# Autodesk Inventor assembly: x_motor
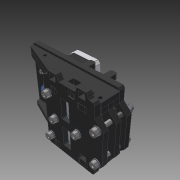
[picture p0: Inventor's stored thumbnail of the model, 180x180]
Saved by Autodesk Inventor 2014 (Build 180170000, 170)
## iProperties
Created: 2014-03-19
Part Number: x_motor
Document SubType Name: Assembly
Designer: buben
Author: buben
## Documents named in this file (18)
- C:\Users\buben\Documents\GitHub\bacon\inventor files\printer parts\6.5 mm\x_motor.iam
- C:\Users\buben\Documents\GitHub\bacon\inventor files\printer parts\6.5 mm\x_motor_back.ipt
- C:\Users\buben\Documents\GitHub\bacon\inventor files\printer parts\6.5 mm\motor_spacer.ipt
- C:\Users\buben\Documents\GitHub\bacon\inventor files\3rd party components\nema_17_stepper\Imported Components\NEMA 17 with T5 Pulley\NEMA 17 with T5 Pulley.iam
- C:\Users\buben\Documents\Inventor\Content Center Files\R2014\en-US\ISO 4762(2)\ISO 4762 - M3 x 16ISO.ipt
- C:\Users\buben\Documents\GitHub\bacon\inventor files\utils\washer_m3.ipt
- C:\Users\buben\Documents\GitHub\bacon\inventor files\printer parts\6.5 mm\x_motor_cable_mount.ipt
- C:\Users\buben\Documents\GitHub\bacon\inventor files\printer parts\6.5 mm\x_motor_cable_mount_brace.ipt
- C:\Users\buben\Documents\GitHub\bacon\inventor files\printer parts\6.5 mm\x_motor_smooth_rod_spacer.ipt
- C:\Users\buben\Documents\GitHub\bacon\inventor files\printer parts\6.5 mm\x_motor_wall_lower.ipt
- C:\Users\buben\Documents\GitHub\bacon\inventor files\printer parts\6.5 mm\x_motor_wall_upper.ipt
- C:\Users\buben\Documents\GitHub\bacon\inventor files\printer parts\6.5 mm\x_motor_middle.ipt
- C:\Users\buben\Documents\GitHub\bacon\inventor files\printer parts\6.5 mm\x_motor_upper_nut_stop.ipt
- C:\Users\buben\Documents\GitHub\bacon\inventor files\3rd party components\linear_bearing_8\Imported Components\LU8MM\LU8MM.iam
- C:\Users\buben\Documents\GitHub\bacon\inventor files\printer parts\6.5 mm\x_motor_top.ipt
- C:\Users\buben\Documents\GitHub\bacon\inventor files\utils\washer_m5.ipt
- C:\Users\buben\Documents\Inventor\Content Center Files\R2014\en-US\ISO 4762(2)\ISO 4762 - M5 x 45ISO.ipt
- C:\Users\buben\Documents\Inventor\Content Center Files\R2014\en-US\ISO 7040\ISO 7040 - M5.ipt
## Components (46 placed, 17 different names)
1. x_motor_back:1 — Mate:4, Tangent:1, Mate:5, Mate:6, Mate:7, Tangent:2, Mate:8, Mate:9, Mate:10, Mate:11, Mate:16, Mate:17, Mate:18, Mate:20, Mate:22, Mate:23, Mate:24, Mate:25, Mate:26, Mate:27, Mate:28, Mate:29, Mate:30, Mate:31, Mate:32, Mate:33, Mate:37, Mate:39, Mate:61, Mate:62, Mate:63, Mate:64, Mate:65, Mate:66
2. motor_spacer:1 — Mate:1, Mate:2, Mate:3, Mate:4, Tangent:1, Tangent:2, Mate:12, Mate:13, Mate:14, Mate:15
3. NEMA 17 with T5 Pulley:1 [sub-assembly] — Mate:1, Mate:2, Mate:3
4. ISO 4762 M3 x 16:1 — Insert:1, Mate:13
5. ISO 4762 M3 x 16:2 — Insert:2, Mate:12
6. ISO 4762 M3 x 16:3 — Insert:3, Mate:15
7. ISO 4762 M3 x 16:4 — Insert:4, Mate:14
8. CSN 02 1702 B B 3,2:1 — Mate:11, Insert:4
9. CSN 02 1702 B B 3,2:2 — Mate:10, Insert:3
10. CSN 02 1702 B B 3,2:3 — Mate:9, Insert:1
11. CSN 02 1702 B B 3,2:4 — Mate:8, Insert:2
12. x_motor_cable_mount:1 — Mate:16, Mate:17, Mate:18, Mate:19, Mate:21
13. x_motor_cable_mount_brace:1 — Mate:19, Mate:20, Mate:21
14. x_motor_smooth_rod_spacer:1 — Mate:23, Mate:24, Mate:27
15. x_motor_smooth_rod_spacer:2 — Mate:22, Mate:25, Mate:26
16. x_motor_wall_lower:1 — Mate:28, Mate:29, Mate:30, Mate:34, Mate:35, Mate:36, Mate:46, Mate:47
17. x_motor_wall_upper:1 — Mate:31, Mate:32, Mate:33, Mate:38
18. x_motor_middle:1 — Mate:34, Mate:35, Mate:36, Mate:40, Mate:41, Mate:42, Mate:43, Mate:44, Mate:45
19. x_motor_upper_nut_stop:1 — Mate:37, Mate:38, Mate:39
20. LU8MM:1 [sub-assembly] — Mate:40, Mate:41, Mate:45, Mate:48
21. LU8MM:2 [sub-assembly] — Mate:42, Mate:43, Mate:44
22. x_motor_top:1 — Mate:46, Mate:47, Mate:48, Mate:49, Mate:50, Mate:51, Mate:52, Mate:53, Mate:54, Mate:55, Mate:56, Mate:57, Mate:58, Mate:59, Mate:60
23. CSN 02 1702 B B 5,3:1 — Mate:53, Mate:56, Insert:9
24. CSN 02 1702 B B 5,3:2 — Mate:51, Mate:57, Insert:7
25. CSN 02 1702 B B 5,3:3 — Mate:50, Mate:59, Insert:5
26. CSN 02 1702 B B 5,3:4 — Mate:49, Mate:60, Insert:6
27. CSN 02 1702 B B 5,3:5 — Mate:52, Mate:58, Insert:8
28. CSN 02 1702 B B 5,3:6 — Mate:54, Mate:55, Insert:10
29. CSN 02 1702 B B 5,3:7 — Mate:64, Mate:70, Mate:79
30. CSN 02 1702 B B 5,3:8 — Mate:65, Mate:71, Mate:83
31. CSN 02 1702 B B 5,3:9 — Mate:66, Mate:72, Mate:81
32. CSN 02 1702 B B 5,3:10 — Mate:63, Mate:69, Mate:77
33. CSN 02 1702 B B 5,3:11 — Mate:61, Mate:67, Mate:75
34. CSN 02 1702 B B 5,3:12 — Mate:62, Mate:68, Mate:73
35. ISO 4762 M5 x 45:1 — Insert:8, Mate:70, Mate:80
36. ISO 4762 M5 x 45:2 — Insert:7, Mate:69, Mate:78
37. ISO 4762 M5 x 45:3 — Insert:5, Mate:72, Mate:82
38. ISO 4762 M5 x 45:4 — Insert:6, Mate:67, Mate:76
39. ISO 4762 M5 x 45:5 — Insert:9, Mate:68, Mate:74
40. ISO 4762 M5 x 45:6 — Insert:10, Mate:71, Mate:84
41. DIN EN ISO 7040 M5:1 — Mate:79, Mate:80
42. DIN EN ISO 7040 M5:2 — Mate:81, Mate:82
43. DIN EN ISO 7040 M5:3 — Mate:83, Mate:84
44. DIN EN ISO 7040 M5:4 — Mate:77, Mate:78
45. DIN EN ISO 7040 M5:5 — Mate:73, Mate:74
46. DIN EN ISO 7040 M5:6 — Mate:75, Mate:76
## Relationships (96: Mate 84, Insert 10, Tangent 2)
- Mate:1: motor_spacer:1 ↔ NEMA 17 with T5 Pulley:1
- Mate:2: motor_spacer:1 ↔ NEMA 17 with T5 Pulley:1
- Mate:3: motor_spacer:1 ↔ NEMA 17 with T5 Pulley:1
- Mate:4: x_motor_back:1 ↔ motor_spacer:1
- Tangent:1: x_motor_back:1 ↔ motor_spacer:1
- Mate:5: x_motor_back:1
- Mate:6: x_motor_back:1
- Mate:7: x_motor_back:1
- Tangent:2: x_motor_back:1 ↔ motor_spacer:1
- Mate:8: x_motor_back:1 ↔ CSN 02 1702 B B 3,2:4
- Mate:9: x_motor_back:1 ↔ CSN 02 1702 B B 3,2:3
- Mate:10: x_motor_back:1 ↔ CSN 02 1702 B B 3,2:2
- Mate:11: x_motor_back:1 ↔ CSN 02 1702 B B 3,2:1
- Insert:1: ISO 4762 M3 x 16:1 ↔ CSN 02 1702 B B 3,2:3
- Insert:2: ISO 4762 M3 x 16:2 ↔ CSN 02 1702 B B 3,2:4
- Insert:3: ISO 4762 M3 x 16:3 ↔ CSN 02 1702 B B 3,2:2
- Insert:4: ISO 4762 M3 x 16:4 ↔ CSN 02 1702 B B 3,2:1
- Mate:12: motor_spacer:1 ↔ ISO 4762 M3 x 16:2
- Mate:13: motor_spacer:1 ↔ ISO 4762 M3 x 16:1
- Mate:14: motor_spacer:1 ↔ ISO 4762 M3 x 16:4
- Mate:15: motor_spacer:1 ↔ ISO 4762 M3 x 16:3
- Mate:16: x_motor_back:1 ↔ x_motor_cable_mount:1
- Mate:17: x_motor_back:1 ↔ x_motor_cable_mount:1
- Mate:18: x_motor_back:1 ↔ x_motor_cable_mount:1
- Mate:19: x_motor_cable_mount:1 ↔ x_motor_cable_mount_brace:1
- Mate:20: x_motor_back:1 ↔ x_motor_cable_mount_brace:1
- Mate:21: x_motor_cable_mount:1 ↔ x_motor_cable_mount_brace:1
- Mate:22: x_motor_back:1 ↔ x_motor_smooth_rod_spacer:2
- Mate:23: x_motor_back:1 ↔ x_motor_smooth_rod_spacer:1
- Mate:24: x_motor_back:1 ↔ x_motor_smooth_rod_spacer:1
- Mate:25: x_motor_back:1 ↔ x_motor_smooth_rod_spacer:2
- Mate:26: x_motor_back:1 ↔ x_motor_smooth_rod_spacer:2
- Mate:27: x_motor_back:1 ↔ x_motor_smooth_rod_spacer:1
- Mate:28: x_motor_back:1 ↔ x_motor_wall_lower:1
- Mate:29: x_motor_back:1 ↔ x_motor_wall_lower:1
- Mate:30: x_motor_back:1 ↔ x_motor_wall_lower:1
- Mate:31: x_motor_back:1 ↔ x_motor_wall_upper:1
- Mate:32: x_motor_back:1 ↔ x_motor_wall_upper:1
- Mate:33: x_motor_back:1 ↔ x_motor_wall_upper:1
- Mate:34: x_motor_wall_lower:1 ↔ x_motor_middle:1
- Mate:35: x_motor_wall_lower:1 ↔ x_motor_middle:1
- Mate:36: x_motor_wall_lower:1 ↔ x_motor_middle:1
- Mate:37: x_motor_back:1 ↔ x_motor_upper_nut_stop:1
- Mate:38: x_motor_wall_upper:1 ↔ x_motor_upper_nut_stop:1
- Mate:39: x_motor_back:1 ↔ x_motor_upper_nut_stop:1
- Mate:40 (7.5 mm): x_motor_middle:1 ↔ LU8MM:1
- Mate:41 (7.5 mm): x_motor_middle:1 ↔ LU8MM:1
- Mate:42 (7.5 mm): x_motor_middle:1 ↔ LU8MM:2
- Mate:43 (7.5 mm): x_motor_middle:1 ↔ LU8MM:2
- Mate:44 (0.5 mm): x_motor_middle:1 ↔ LU8MM:2
- Mate:45 (0.5 mm): x_motor_middle:1 ↔ LU8MM:1
- Mate:46: x_motor_wall_lower:1 ↔ x_motor_top:1
- Mate:47: x_motor_wall_lower:1 ↔ x_motor_top:1
- Mate:48 (7.5 mm): LU8MM:1 ↔ x_motor_top:1
- Mate:49: x_motor_top:1 ↔ CSN 02 1702 B B 5,3:4
- Mate:50: x_motor_top:1 ↔ CSN 02 1702 B B 5,3:3
- Mate:51: x_motor_top:1 ↔ CSN 02 1702 B B 5,3:2
- Mate:52: x_motor_top:1 ↔ CSN 02 1702 B B 5,3:5
- Mate:53: x_motor_top:1 ↔ CSN 02 1702 B B 5,3:1
- Mate:54: x_motor_top:1 ↔ CSN 02 1702 B B 5,3:6
- Mate:55: x_motor_top:1 ↔ CSN 02 1702 B B 5,3:6
- Mate:56: x_motor_top:1 ↔ CSN 02 1702 B B 5,3:1
- Mate:57: x_motor_top:1 ↔ CSN 02 1702 B B 5,3:2
- Mate:58: x_motor_top:1 ↔ CSN 02 1702 B B 5,3:5
- Mate:59: x_motor_top:1 ↔ CSN 02 1702 B B 5,3:3
- Mate:60: x_motor_top:1 ↔ CSN 02 1702 B B 5,3:4
- Insert:5: CSN 02 1702 B B 5,3:3 ↔ ISO 4762 M5 x 45:3
- Insert:6: CSN 02 1702 B B 5,3:4 ↔ ISO 4762 M5 x 45:4
- Insert:7: CSN 02 1702 B B 5,3:2 ↔ ISO 4762 M5 x 45:2
- Insert:8: CSN 02 1702 B B 5,3:5 ↔ ISO 4762 M5 x 45:1
- Insert:9: CSN 02 1702 B B 5,3:1 ↔ ISO 4762 M5 x 45:5
- Insert:10: CSN 02 1702 B B 5,3:6 ↔ ISO 4762 M5 x 45:6
- Mate:61: x_motor_back:1 ↔ CSN 02 1702 B B 5,3:11
- Mate:62: x_motor_back:1 ↔ CSN 02 1702 B B 5,3:12
- Mate:63: x_motor_back:1 ↔ CSN 02 1702 B B 5,3:10
- Mate:64: x_motor_back:1 ↔ CSN 02 1702 B B 5,3:7
- Mate:65: x_motor_back:1 ↔ CSN 02 1702 B B 5,3:8
- Mate:66: x_motor_back:1 ↔ CSN 02 1702 B B 5,3:9
- Mate:67: CSN 02 1702 B B 5,3:11 ↔ ISO 4762 M5 x 45:4
- Mate:68: CSN 02 1702 B B 5,3:12 ↔ ISO 4762 M5 x 45:5
- Mate:69: CSN 02 1702 B B 5,3:10 ↔ ISO 4762 M5 x 45:2
- Mate:70: CSN 02 1702 B B 5,3:7 ↔ ISO 4762 M5 x 45:1
- Mate:71: CSN 02 1702 B B 5,3:8 ↔ ISO 4762 M5 x 45:6
- Mate:72: CSN 02 1702 B B 5,3:9 ↔ ISO 4762 M5 x 45:3
- Mate:73: CSN 02 1702 B B 5,3:12 ↔ DIN EN ISO 7040 M5:5
- Mate:74: ISO 4762 M5 x 45:5 ↔ DIN EN ISO 7040 M5:5
- Mate:75: CSN 02 1702 B B 5,3:11 ↔ DIN EN ISO 7040 M5:6
- Mate:76: ISO 4762 M5 x 45:4 ↔ DIN EN ISO 7040 M5:6
- Mate:77: CSN 02 1702 B B 5,3:10 ↔ DIN EN ISO 7040 M5:4
- Mate:78: ISO 4762 M5 x 45:2 ↔ DIN EN ISO 7040 M5:4
- Mate:79: CSN 02 1702 B B 5,3:7 ↔ DIN EN ISO 7040 M5:1
- Mate:80: ISO 4762 M5 x 45:1 ↔ DIN EN ISO 7040 M5:1
- Mate:81: CSN 02 1702 B B 5,3:9 ↔ DIN EN ISO 7040 M5:2
- Mate:82: ISO 4762 M5 x 45:3 ↔ DIN EN ISO 7040 M5:2
- Mate:83: CSN 02 1702 B B 5,3:8 ↔ DIN EN ISO 7040 M5:3
- Mate:84: ISO 4762 M5 x 45:6 ↔ DIN EN ISO 7040 M5:3
